# Autodesk Inventor assembly: Hamdle Assembly
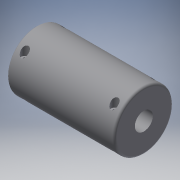
[picture p0: Inventor's stored thumbnail of the model, 180x180]
Saved by Autodesk Inventor 2018 (Build 220112000, 112)
## iProperties
Created: 2018-01-14
Part Number: Hamdle Assembly
Document SubType Name: Assembly
Designer: prakh
Author: prakh
## Documents named in this file (5)
- D:\GIT\ModernMobility\CADS\Handle CADs\Hamdle Assembly.iam
- D:\GIT\ModernMobility\CADS\Handle CADs\Slider Mount_A.ipt
- D:\GIT\ModernMobility\CADS\Handle CADs\Slider Mount_B.ipt
- D:\GIT\ModernMobility\CADS\Handle CADs\Slider Mount_C.ipt
- D:\GIT\ModernMobility\CADS\Handle CADs\Slider Mount_D.ipt
## Components (4 placed, 4 different names)
1. Slider Mount_A:1 — Mate:1, Mate:2, Flush:1, Mate:3
2. Slider Mount_B:1 — Mate:1, Mate:2, Flush:1, Mate:4
3. Slider Mount_C:1 — Mate:3, Mate:4, Mate:5, Flush:2
4. Slider Mount_D:1 — Mate:5, Flush:2
## Relationships (7: Mate 5, Flush 2)
- Mate:1: Slider Mount_A:1 ↔ Slider Mount_B:1
- Mate:2: Slider Mount_A:1 ↔ Slider Mount_B:1
- Flush:1: Slider Mount_A:1 ↔ Slider Mount_B:1
- Mate:3: Slider Mount_A:1 ↔ Slider Mount_C:1
- Mate:4: Slider Mount_B:1 ↔ Slider Mount_C:1
- Mate:5: Slider Mount_C:1 ↔ Slider Mount_D:1
- Flush:2: Slider Mount_C:1 ↔ Slider Mount_D:1
